# Autodesk Inventor assembly: fixer
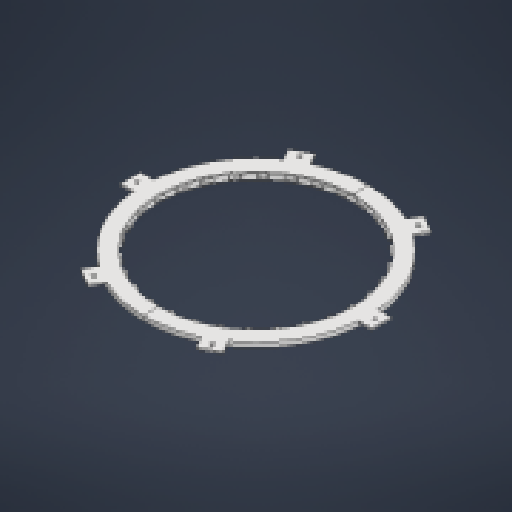
[picture p0: Inventor's stored thumbnail of the model, 512x512]
Saved by Autodesk Inventor 2026.1 (Build 301233020, 233B)
## iProperties
Created: 2025-12-01
Part Number: fixer
Document SubType Name: Assembly
Designer: jaewook
Author: jaewook
## Documents named in this file (4)
- C:\Users\kjh19\Documents\Inventor\project\final\fixer.iam
- C:\Users\kjh19\Documents\Inventor\project\final\fixer_1.ipt
- C:\Users\kjh19\Documents\Inventor\project\final\fixer_left_v1.ipt
- C:\Users\kjh19\Documents\Inventor\project\final\fixer_right_v1.ipt
## Components (3 placed, 3 different names)
1. fixer_1:1
2. fixer_left_v1:1 — 메이트:1, 메이트:2, 메이트:3
3. fixer_right_v1:1 — 메이트:1, 메이트:2, 메이트:3
## Relationships (3: Mate 3)
- 메이트:1 [Mate]: fixer_left_v1:1 ↔ fixer_right_v1:1
- 메이트:2 [Mate]: fixer_left_v1:1 ↔ fixer_right_v1:1
- 메이트:3 [Mate]: fixer_left_v1:1 ↔ fixer_right_v1:1
